# Autodesk Inventor assembly: Assembly1
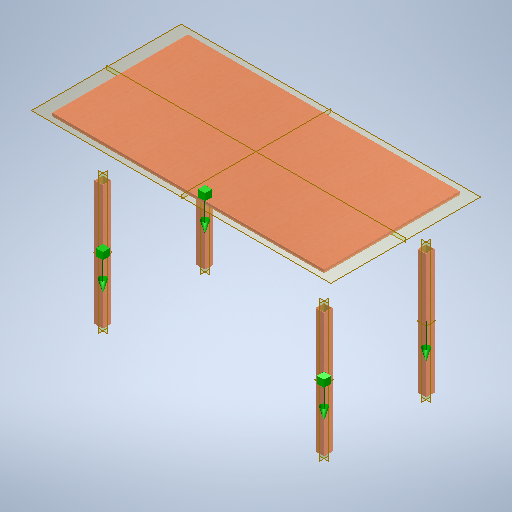
[picture p0: Inventor's stored thumbnail of the model, 512x512]
Saved by Autodesk Inventor 2025.2 (Build 292293000, 293)
## iProperties
Created: 2025-04-02
Part Number: Assembly1
Document SubType Name: Assembly
Designer: kenne
Author: kenne
## Documents named in this file (3)
- C:\Users\kenne\OneDrive\Ambiente de Trabalho\Robotica & Automação\Sistemas de Microcontroladores\Learning\Inventor\Exercices\Mesa_ergo\Assembly1.iam
- C:\Users\kenne\OneDrive\Ambiente de Trabalho\Robotica & Automação\Sistemas de Microcontroladores\Learning\Inventor\Exercices\Mesa_ergo\Tampo.ipt
- C:\Users\kenne\OneDrive\Ambiente de Trabalho\Robotica & Automação\Sistemas de Microcontroladores\Learning\Inventor\Exercices\Mesa_ergo\perna.ipt
## Components (5 placed, 2 different names)
1. Tampo:1 — Flush:1, Flush:2, Flush:3, Mate:1, Flush:4, Flush:5, Mate:4, Mate:6, Flush:10
2. perna:1 — Mate:1, Flush:4, Flush:5, Flush:6, Flush:7, Mate:2, Flush:8, Mate:3, Flush:9
3. perna:2 — Flush:7, Mate:2, Mate:5, Mate:6
4. perna:3 — Flush:9, Mate:5, Flush:10
5. perna:4 — Flush:6, Flush:8, Mate:3, Mate:4
## Relationships (16: Flush 10, Mate 6)
- Flush:1: Tampo:1
- Flush:2: Tampo:1
- Flush:3: Tampo:1
- Mate:1: Tampo:1 ↔ perna:1
- Flush:4 (-300 mm): Tampo:1 ↔ perna:1
- Flush:5 (-700 mm): Tampo:1 ↔ perna:1
- Flush:6: perna:1 ↔ perna:4
- Flush:7: perna:1 ↔ perna:2
- Mate:2: perna:1 ↔ perna:2
- Flush:8: perna:1 ↔ perna:4
- Mate:3: perna:1 ↔ perna:4
- Flush:9: perna:1 ↔ perna:3
- Mate:4 (-300 mm): Tampo:1 ↔ perna:4
- Mate:5 (600 mm): perna:2 ↔ perna:3
- Mate:6 (-600 mm): Tampo:1 ↔ perna:2
- Flush:10 (600 mm): Tampo:1 ↔ perna:3
